# Autodesk Inventor assembly: FE-00006
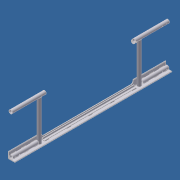
[picture p0: Inventor's stored thumbnail of the model, 180x180]
Saved by Autodesk Inventor 2012 (Build 160160000, 160)
## iProperties
Company: FIRST
Created: 2008-05-25
Part Number: FE-00006
Document SubType Name: Weldment
Designer: DFOSTER
Description: FIELD RAIL GATE - ASSEMBLY
Weld Material: Welded Aluminum-6061
Title: FIELD RAIL GATE - ASSEMBLY
Author: DFOSTER
## Documents named in this file (8)
- C:\Data Folder\FRC 2012 Field\Components\FE-00006.iam
- C:\Data Folder\FRC 2012 Field\Components\FE-00006-01.ipt
- C:\Data Folder\FRC 2012 Field\Components\FE-00006-02.ipt
- C:\Data Folder\FRC 2012 Field\Components\FE-00006-09.ipt
- C:\Data Folder\FRC 2012 Field\Components\FE-00006-10.ipt
- C:\Data Folder\FRC 2012 Field\Components\FE-00006-03.ipt
- C:\Data Folder\FRC 2012 Field\Components\FE-00006-05.ipt
- C:\Data Folder\FRC 2012 Field\Components\FE-00006-08.ipt
## Components (9 placed, 7 different names)
1. FE-00006-01:1 — Tangent:1, Tangent:2, Flush:1, Angle:1, Tangent:3, Tangent:4, Flush:2, Angle:2, Mate:1, Mate:2, Flush:3, Mate:3, Mate:4, Tangent:5, Tangent:8, Flush:4, Angle:5, Angle:7, Angle:8, Mate:16, Mate:17
2. FE-00006-02:1 — Tangent:1, Tangent:2, Flush:1, Angle:1, Angle:3
3. FE-00006-02:2 — Tangent:3, Tangent:4, Flush:2, Angle:2, Angle:4
4. FE-00006-09:1 — Mate:1, Mate:2, Flush:3
5. FE-00006-10:1 — Mate:3, Mate:5, Tangent:8, Angle:4, Mate:6, Mate:17
6. FE-00006-10:2 — Mate:4, Mate:5, Tangent:5, Angle:3, Mate:7, Mate:16
7. FE-00006-03:1 — Mate:6, Mate:14, Mate:15, Flush:5, Angle:8
8. FE-00006-05:1 — Flush:4, Mate:7, Angle:5, Mate:14
9. FE-00006-08:1 — Mate:15, Flush:5, Angle:7
## Relationships (29: Mate 11, Angle 7, Tangent 6, Flush 5)
- Tangent:1: FE-00006-01:1 ↔ FE-00006-02:1
- Tangent:2: FE-00006-01:1 ↔ FE-00006-02:1
- Flush:1 (6.35 mm): FE-00006-01:1 ↔ FE-00006-02:1
- Angle:1 (90 deg): FE-00006-01:1 ↔ FE-00006-02:1
- Tangent:3: FE-00006-01:1 ↔ FE-00006-02:2
- Tangent:4: FE-00006-01:1 ↔ FE-00006-02:2
- Flush:2 (6.35 mm): FE-00006-01:1 ↔ FE-00006-02:2
- Angle:2 (-90 deg): FE-00006-01:1 ↔ FE-00006-02:2
- Mate:1: FE-00006-01:1 ↔ FE-00006-09:1
- Mate:2 (6.35 mm): FE-00006-01:1 ↔ FE-00006-09:1
- Flush:3 (381 mm): FE-00006-01:1 ↔ FE-00006-09:1
- Mate:3: FE-00006-01:1 ↔ FE-00006-10:1
- Mate:4: FE-00006-01:1 ↔ FE-00006-10:2
- Mate:5: FE-00006-10:1 ↔ FE-00006-10:2
- Tangent:5: FE-00006-01:1 ↔ FE-00006-10:2
- Tangent:8: FE-00006-01:1 ↔ FE-00006-10:1
- Angle:3 (180 deg): FE-00006-02:1 ↔ FE-00006-10:2
- Angle:4 (0 deg): FE-00006-02:2 ↔ FE-00006-10:1
- Mate:6: FE-00006-10:1 ↔ FE-00006-03:1
- Flush:4: FE-00006-01:1 ↔ FE-00006-05:1
- Mate:7: FE-00006-10:2 ↔ FE-00006-05:1
- Angle:5 (-90 deg): FE-00006-01:1 ↔ FE-00006-05:1
- Mate:14 (-1828.8 mm): FE-00006-03:1 ↔ FE-00006-05:1
- Mate:15: FE-00006-03:1 ↔ FE-00006-08:1
- Flush:5 (-12.7 mm): FE-00006-03:1 ↔ FE-00006-08:1
- Angle:7 (0 deg): FE-00006-01:1 ↔ FE-00006-08:1
- Angle:8 (-90 deg): FE-00006-01:1 ↔ FE-00006-03:1
- Mate:16 (-332.5813 mm): FE-00006-01:1 ↔ FE-00006-10:2
- Mate:17 (-332.5813 mm): FE-00006-01:1 ↔ FE-00006-10:1
